# Autodesk Inventor assembly: Imm_mount_ver1
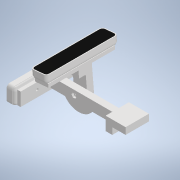
[picture p0: Inventor's stored thumbnail of the model, 180x180]
Saved by Autodesk Inventor 2022 (Build 260153000, 153)
## iProperties
Created: 2021-10-08
Part Number: Imm_mount_ver1
Document SubType Name: Assembly
Designer: skcre
Author: skcre
## Documents named in this file (4)
- D:\Documents\Inventor\ARRF\jetson_cv_hub_ver1\Imm_mount_ver1.iam
- D:\Documents\Inventor\ARRF\jetson_cv_hub_ver1\t265_mount_imm.ipt
- D:\Documents\Inventor\ARRF\jetson_cv_hub_ver1\t265_mount_imm_secondary.ipt
- D:\Documents\Inventor\ARRF\jetson_cv_hub_ver1\External_models\t265ass_Simplify_1.ipt
## Components (4 placed, 3 different names)
1. t265_mount_imm:1 — Mate:1, Mate:2, Mate:3, Mate:4, Mate:5
2. t265_mount_imm_secondary:1 — Mate:1, Mate:2, Mate:6, Mate:7, Mate:8
3. t265ass_Simplify_1:1 — Mate:3, Mate:4, Mate:5
4. t265ass_Simplify_1:2 — Mate:6, Mate:7, Mate:8
## Relationships (8: Mate 8)
- Mate:1: t265_mount_imm:1 ↔ t265_mount_imm_secondary:1
- Mate:2: t265_mount_imm:1 ↔ t265_mount_imm_secondary:1
- Mate:3: t265_mount_imm:1 ↔ t265ass_Simplify_1:1
- Mate:4: t265_mount_imm:1 ↔ t265ass_Simplify_1:1
- Mate:5: t265_mount_imm:1 ↔ t265ass_Simplify_1:1
- Mate:6: t265_mount_imm_secondary:1 ↔ t265ass_Simplify_1:2
- Mate:7: t265_mount_imm_secondary:1 ↔ t265ass_Simplify_1:2
- Mate:8: t265_mount_imm_secondary:1 ↔ t265ass_Simplify_1:2
